# Autodesk Inventor assembly: Zespół1
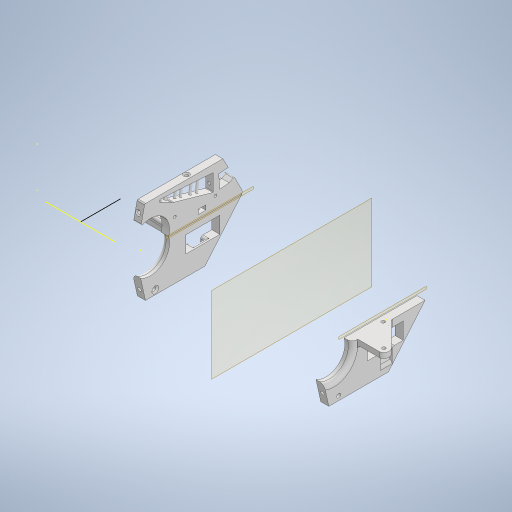
[picture p0: Inventor's stored thumbnail of the model, 512x512]
Saved by Autodesk Inventor 2023 (Build 270158000, 158)
## iProperties
Created: 2023-04-14
Part Number: Zespół1
Document SubType Name: Assembly
Designer: Kamil
Author: Kamil
## Documents named in this file (4)
- C:\Users\Kamil\Desktop\MojeRoboty\Stefan\mechanics\Zespół1.iam
- C:\Users\Kamil\Desktop\MojeRoboty\Stefan\mechanics\sciana_prawa_v4.ipt
- C:\Users\Kamil\Desktop\MojeRoboty\Stefan\mechanics\sciana PRE 2.0.ipt
- C:\Users\Kamil\Desktop\MojeRoboty\Stefan\mechanics\sciana PRE 2.0_MIR1.ipt
## Components (3 placed, 3 different names)
1. sciana_prawa_v4:1 — Zestawiające:1, Równoległe:1, Zestawiające:2
2. sciana PRE 2.0:1 — Zestawiające:1, Równoległe:1, Zestawiające:2, Równoległe:2
3. sciana PRE 2.0_MIR1:1 — Zestawiające:3
## Relationships (5: Mate 3, Flush 2)
- Zestawiające:1 [Mate]: sciana_prawa_v4:1 ↔ sciana PRE 2.0:1
- Równoległe:1 [Flush]: sciana_prawa_v4:1 ↔ sciana PRE 2.0:1
- Zestawiające:2 [Mate]: sciana_prawa_v4:1 ↔ sciana PRE 2.0:1
- Równoległe:2 [Flush] (76.2 mm): sciana PRE 2.0:1
- Zestawiające:3 [Mate] (76.2 mm): sciana PRE 2.0_MIR1:1
